# Autodesk Inventor assembly: load_cell_dowel_pin_screw
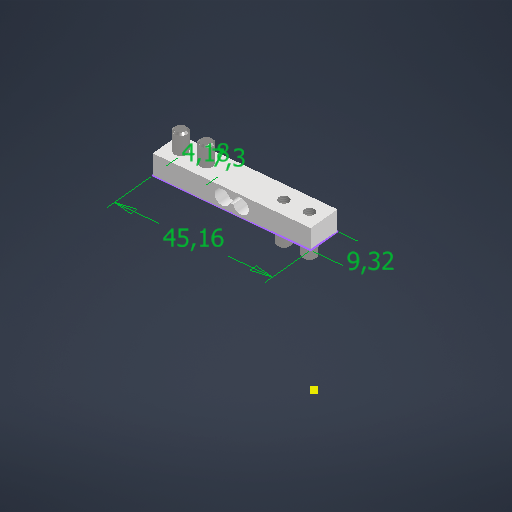
[picture p0: Inventor's stored thumbnail of the model, 512x512]
Saved by Autodesk Inventor 2026 (Build 300175000, 175)
## iProperties
Created: 2025-04-21
Part Number: load_cell_dowel_pin_screw
Document SubType Name: Assembly
Designer: Paul Juschitz
Author: Paul Juschitz
## Documents named in this file (3)
- C:\Users\Paul Juschitz\Documents\private\m5_GBW_mod\M5_GBW_mod\CAD\load_cell_dowel_pin_screw.iam
- C:\Users\Paul Juschitz\Documents\private\m5_GBW_mod\M5_GBW_mod\CAD\load_cell.ipt
- C:\Users\Paul Juschitz\Documents\Inventor\Content Center Files\R2026\en-US\DIN 927\DIN 927 - M3 x 6-14H.ipt
## Components (5 placed, 2 different names)
1. load_cell:1 — Angle:1, Cylindrical:1, Cylindrical:2, Cylindrical:3, Cylindrical:4, Mate:1, Mate:2, Mate:3, Mate:4
2. DIN 927 M3 x 6-14H:1 — Cylindrical:2, Mate:1
3. DIN 927 M3 x 6-14H:2 — Cylindrical:1, Mate:2
4. DIN 927 M3 x 6-14H:3 — Cylindrical:3, Mate:3
5. DIN 927 M3 x 6-14H:4 — Cylindrical:4, Mate:4
## Relationships (9: CylindricalJoint 4, Mate 4, Angle 1)
- Angle:1 (0 deg): load_cell:1
- Cylindrical:1: load_cell:1 ↔ DIN 927 M3 x 6-14H:2
- Cylindrical:2: load_cell:1 ↔ DIN 927 M3 x 6-14H:1
- Cylindrical:3: load_cell:1 ↔ DIN 927 M3 x 6-14H:3
- Cylindrical:4: load_cell:1 ↔ DIN 927 M3 x 6-14H:4
- Mate:1: load_cell:1 ↔ DIN 927 M3 x 6-14H:1
- Mate:2: load_cell:1 ↔ DIN 927 M3 x 6-14H:2
- Mate:3: load_cell:1 ↔ DIN 927 M3 x 6-14H:3
- Mate:4: load_cell:1 ↔ DIN 927 M3 x 6-14H:4
